# Autodesk Inventor assembly: Chasis Montaje
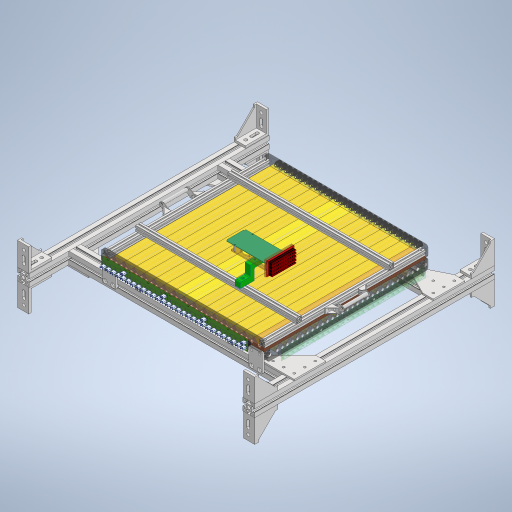
[picture p0: Inventor's stored thumbnail of the model, 512x512]
Saved by Autodesk Inventor 2024.2 (Build 282272000, 272)
## iProperties
Created: 2025-06-05
Part Number: Chasis Montaje
Document SubType Name: Assembly
Designer: ja.restrepo1
Author: ja.restrepo1
## Documents named in this file (4)
- I:\MICROMECANICA\ALTAS ENERGIAS\Deteccion de Muones\Detectores centelladores\Partes Detector Centellador\SE Chasis DC\SE Chasis Montaje.iam
- I:\MICROMECANICA\ALTAS ENERGIAS\Deteccion de Muones\Detectores centelladores\Partes Detector Centellador\SE Matriz Centelladora DC\SE Matriz Centelladora DC.iam
- I:\MICROMECANICA\ALTAS ENERGIAS\Deteccion de Muones\Detectores centelladores\Partes Detector Centellador\SE Base Matriz Centelladora DC\SE Base Matriz Centelladora DC.iam
- I:\MICROMECANICA\ALTAS ENERGIAS\Deteccion de Muones\Detectores centelladores\Partes Detector Centellador\SE Chasis DC\Partes Chasis DC\Soporte Montaje Matriz Centelladora.ipt
## Components (6 placed, 3 different names)
1. SE Matriz Centelladora DC:1 [sub-assembly] — Nivelación:1, Nivelación:2, Nivelación:3, Coincidencia:1, Coincidencia:2, Coincidencia:3, Coincidencia:4, Coincidencia:5, Coincidencia:6, Coincidencia:7, Coincidencia:8, Coincidencia:9
2. SE Base Matriz Centelladora DC:1 [sub-assembly] — Coincidencia:10, Coincidencia:11
3. Soporte Montaje Matriz Centelladora:1 — Coincidencia:9, Nivelación:6, Nivelación:7
4. Soporte Montaje Matriz Centelladora:2 — Nivelación:4, Nivelación:5, Coincidencia:8, Coincidencia:10, Coincidencia:11
5. Soporte Montaje Matriz Centelladora:3 — Coincidencia:2, Coincidencia:4, Coincidencia:7, Nivelación:4, Nivelación:5
6. Soporte Montaje Matriz Centelladora:4 — Coincidencia:3, Coincidencia:5, Coincidencia:6, Nivelación:6, Nivelación:7
## Relationships (18: Mate 11, Flush 7)
- Nivelación:1 [Flush]: SE Matriz Centelladora DC:1
- Nivelación:2 [Flush]: SE Matriz Centelladora DC:1
- Nivelación:3 [Flush]: SE Matriz Centelladora DC:1
- Coincidencia:1 [Mate]: SE Matriz Centelladora DC:1
- Coincidencia:2 [Mate]: SE Matriz Centelladora DC:1 ↔ Soporte Montaje Matriz Centelladora:3
- Coincidencia:3 [Mate]: SE Matriz Centelladora DC:1 ↔ Soporte Montaje Matriz Centelladora:4
- Coincidencia:4 [Mate]: SE Matriz Centelladora DC:1 ↔ Soporte Montaje Matriz Centelladora:3
- Coincidencia:5 [Mate]: SE Matriz Centelladora DC:1 ↔ Soporte Montaje Matriz Centelladora:4
- Coincidencia:6 [Mate] (2 mm): SE Matriz Centelladora DC:1 ↔ Soporte Montaje Matriz Centelladora:4
- Coincidencia:7 [Mate] (2 mm): SE Matriz Centelladora DC:1 ↔ Soporte Montaje Matriz Centelladora:3
- Nivelación:4 [Flush]: Soporte Montaje Matriz Centelladora:2 ↔ Soporte Montaje Matriz Centelladora:3
- Nivelación:5 [Flush]: Soporte Montaje Matriz Centelladora:2 ↔ Soporte Montaje Matriz Centelladora:3
- Coincidencia:8 [Mate]: SE Matriz Centelladora DC:1 ↔ Soporte Montaje Matriz Centelladora:2
- Coincidencia:9 [Mate]: SE Matriz Centelladora DC:1 ↔ Soporte Montaje Matriz Centelladora:1
- Nivelación:6 [Flush]: Soporte Montaje Matriz Centelladora:1 ↔ Soporte Montaje Matriz Centelladora:4
- Nivelación:7 [Flush]: Soporte Montaje Matriz Centelladora:1 ↔ Soporte Montaje Matriz Centelladora:4
- Coincidencia:10 [Mate]: SE Base Matriz Centelladora DC:1 ↔ Soporte Montaje Matriz Centelladora:2
- Coincidencia:11 [Mate]: SE Base Matriz Centelladora DC:1 ↔ Soporte Montaje Matriz Centelladora:2
